# Autodesk Inventor assembly: bottomLayer
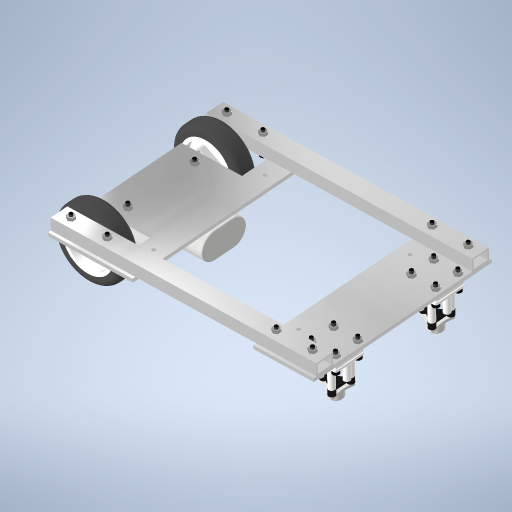
[picture p0: Inventor's stored thumbnail of the model, 512x512]
Saved by Autodesk Inventor 2024 (Build 280153000, 153)
## iProperties
Created: 2023-10-26
Part Number: bottomLayer
Document SubType Name: Assembly
Designer: jwith
Mass: 389.888 g
Surface Area: 1411.33 cm^2
Volume: 227.835 cm^3
Density: 1.71127 g/cm^3
Author: jwith
## Documents named in this file (14)
- C:\Users\jwith\OneDrive\kikaiken\inventor\general-useLandRobotV1\bottomLayer.iam
- C:\Users\jwith\OneDrive\kikaiken\inventor\general-useLandRobotV1\backPlate.ipt
- C:\Users\jwith\OneDrive\kikaiken\inventor\general-useLandRobotV1\frontPlate.ipt
- C:\Users\jwith\OneDrive\kikaiken\inventor\general-useLandRobotV1\right_ASP.ipt
- C:\Users\jwith\OneDrive\kikaiken\inventor\general-useLandRobotV1\left_ASP.ipt
- C:\Users\jwith\OneDrive\kikaiken\inventor\general-useLandRobotV1\Content Center Files\R2024\ja-JP\SpringWasher\SpringWasher_3007SL.ipt
- C:\Users\jwith\OneDrive\kikaiken\inventor\general-useLandRobotV1\Content Center Files\R2024\ja-JP\HexSocketCapScrew\HexSocketCapScrew_3005018BK.ipt
- C:\Users\jwith\OneDrive\kikaiken\inventor\general-useLandRobotV1\Content Center Files\R2024\ja-JP\HexNut_Type1\HexNut_Type1_30050SL.ipt
- C:\Users\jwith\OneDrive\kikaiken\inventor\general-useLandRobotV1\資料\車体設計例\plate_5mm.ipt
- C:\Users\jwith\OneDrive\kikaiken\inventor\general-useLandRobotV1\資料\車体設計例\TAMIYA_ballcaster_35mm.iam
- C:\Users\jwith\OneDrive\kikaiken\inventor\general-useLandRobotV1\Content Center Files\R2024\ja-JP\HexSocketCapScrew\HexSocketCapScrew_3005015BK.ipt
- C:\Users\jwith\OneDrive\kikaiken\inventor\general-useLandRobotV1\資料\車体設計例\TAMIYA_DoubleGearBox.iam
- C:\Users\jwith\OneDrive\kikaiken\inventor\general-useLandRobotV1\Content Center Files\R2024\ja-JP\HexSocketCapScrew\HexSocketCapScrew_3005010BK.ipt
- C:\Users\jwith\OneDrive\kikaiken\inventor\general-useLandRobotV1\資料\車体設計例\ナロータイヤセット.iam
## Components (56 placed, 13 different names)
1. backPlate:1 — 回転:25, メイト:68, 回転:26, 回転:27, 回転:28, 回転:29, 回転:30, メイト:69, メイト:70, メイト:71, メイト:73, メイト:74, メイト:75, メイト:80, メイト:81, メイト:82, メイト:83, メイト:85, メイト:86, メイト:87
2. frontPlate:1 — 回転:1, 回転:2, 回転:5, 回転:6, メイト:1, メイト:2, メイト:3, メイト:5, メイト:6, メイト:7, メイト:25, メイト:26, メイト:27, メイト:29, メイト:30, メイト:31, 回転:9, 回転:10, 回転:11, 回転:12, 回転:13, 回転:14, 回転:15, 回転:16, メイト:36, メイト:40, メイト:44, メイト:48, メイト:52, メイト:56, メイト:60, メイト:64
3. right_ASP:1 — 回転:5, 回転:6, メイト:28, メイト:32, 回転:26, 回転:27, メイト:72, メイト:76
4. left_ASP:1 — 回転:1, 回転:2, メイト:4, メイト:8, 回転:28, 回転:29, メイト:84, メイト:88
5. SpringWasher M3-1.1:1 — メイト:1, メイト:2, 挿入:1
6. HexSocketCapScrew M3x0.5-18:1 — 挿入:1
7. HexNut_Type1 M3x0.5:1 — メイト:3, メイト:4
8. SpringWasher M3-1.1:2 — メイト:5, メイト:6, 挿入:2
9. HexSocketCapScrew M3x0.5-18:2 — 挿入:2
10. HexNut_Type1 M3x0.5:2 — メイト:7, メイト:8
11. SpringWasher M3-1.1:7 — メイト:25, メイト:26, 挿入:7
12. HexSocketCapScrew M3x0.5-18:7 — 挿入:7
13. HexNut_Type1 M3x0.5:7 — メイト:27, メイト:28
14. SpringWasher M3-1.1:8 — メイト:29, メイト:30, 挿入:8
15. HexSocketCapScrew M3x0.5-18:8 — 挿入:8
16. HexNut_Type1 M3x0.5:8 — メイト:31, メイト:32
17. plate_5mm:1 — 回転:13, 回転:14, 回転:15, 回転:16, 回転:21, 回転:22, 回転:23, 回転:24
18. plate_5mm:2 — 回転:9, 回転:10, 回転:11, 回転:12, 回転:17, 回転:18, 回転:19, 回転:20, メイト:33, メイト:35, メイト:45, メイト:47
19. TAMIYA_ballcaster_35mm:1 [sub-assembly] — 回転:17, 回転:18, 回転:19, 回転:20, メイト:34, メイト:37, メイト:38, メイト:39, メイト:41, メイト:42, メイト:43, メイト:46
20. TAMIYA_ballcaster_35mm:2 [sub-assembly] — 回転:21, 回転:22, 回転:23, 回転:24, メイト:49, メイト:50, メイト:51, メイト:53, メイト:54, メイト:55, メイト:57, メイト:58, メイト:59, メイト:61, メイト:62, メイト:63
21. HexSocketCapScrew M3x0.5-15:1 — メイト:33, メイト:34
22. HexNut_Type1 M3x0.5:9 — メイト:35, メイト:36
23. HexSocketCapScrew M3x0.5-15:2 — メイト:37, メイト:38
24. HexNut_Type1 M3x0.5:10 — メイト:39, メイト:40
25. HexSocketCapScrew M3x0.5-15:3 — メイト:41, メイト:42
26. HexNut_Type1 M3x0.5:11 — メイト:43, メイト:44
27. HexSocketCapScrew M3x0.5-15:4 — メイト:45, メイト:46
28. HexNut_Type1 M3x0.5:12 — メイト:47, メイト:48
29. HexSocketCapScrew M3x0.5-15:5 — メイト:49, メイト:50
30. HexNut_Type1 M3x0.5:13 — メイト:51, メイト:52
31. HexSocketCapScrew M3x0.5-15:6 — メイト:53, メイト:54
32. HexNut_Type1 M3x0.5:14 — メイト:55, メイト:56
33. HexSocketCapScrew M3x0.5-15:7 — メイト:57, メイト:58
34. HexNut_Type1 M3x0.5:15 — メイト:59, メイト:60
35. HexSocketCapScrew M3x0.5-15:8 — メイト:61, メイト:62
36. HexNut_Type1 M3x0.5:16 — メイト:63, メイト:64
37. TAMIYA_DoubleGearBox:1 [sub-assembly] — 回転:25, メイト:65, メイト:66, メイト:67, リジッド:1, 回転:30, メイト:77, メイト:78, メイト:79, リジッド:2
38. HexSocketCapScrew M3x0.5-10:1 — メイト:65, メイト:66
39. HexNut_Type1 M3x0.5:17 — メイト:67, メイト:68
40. ナロータイヤセット:1 [sub-assembly] — リジッド:1
41. SpringWasher M3-1.1:9 — メイト:69, メイト:70, 挿入:9
42. HexSocketCapScrew M3x0.5-18:9 — 挿入:9
43. HexNut_Type1 M3x0.5:18 — メイト:71, メイト:72
44. SpringWasher M3-1.1:10 — メイト:73, メイト:74, 挿入:10
45. HexSocketCapScrew M3x0.5-18:10 — 挿入:10
46. HexNut_Type1 M3x0.5:19 — メイト:75, メイト:76
47. SpringWasher M3-1.1:11 — メイト:77, メイト:78, 挿入:11
48. HexSocketCapScrew M3x0.5-10:2 — 挿入:11
49. HexNut_Type1 M3x0.5:20 — メイト:79, メイト:80
50. SpringWasher M3-1.1:12 — メイト:81, メイト:82, 挿入:12
51. HexSocketCapScrew M3x0.5-18:11 — 挿入:12
52. HexNut_Type1 M3x0.5:21 — メイト:83, メイト:84
53. SpringWasher M3-1.1:13 — メイト:85, メイト:86, 挿入:13
54. HexSocketCapScrew M3x0.5-18:12 — 挿入:13
55. HexNut_Type1 M3x0.5:22 — メイト:87, メイト:88
56. ナロータイヤセット:2 [sub-assembly] — リジッド:2
## Relationships (109: Mate 72, RevoluteJoint 26, Insert 9, WeldJoint 2)
- 回転:1 [RevoluteJoint]: frontPlate:1 ↔ left_ASP:1
- 回転:2 [RevoluteJoint]: frontPlate:1 ↔ left_ASP:1
- 回転:5 [RevoluteJoint]: frontPlate:1 ↔ right_ASP:1
- 回転:6 [RevoluteJoint]: frontPlate:1 ↔ right_ASP:1
- メイト:1 [Mate]: frontPlate:1 ↔ SpringWasher M3-1.1:1
- メイト:2 [Mate]: frontPlate:1 ↔ SpringWasher M3-1.1:1
- 挿入:1 [Insert]: SpringWasher M3-1.1:1 ↔ HexSocketCapScrew M3x0.5-18:1
- メイト:3 [Mate]: frontPlate:1 ↔ HexNut_Type1 M3x0.5:1
- メイト:4 [Mate]: left_ASP:1 ↔ HexNut_Type1 M3x0.5:1
- メイト:5 [Mate]: frontPlate:1 ↔ SpringWasher M3-1.1:2
- メイト:6 [Mate]: frontPlate:1 ↔ SpringWasher M3-1.1:2
- 挿入:2 [Insert]: SpringWasher M3-1.1:2 ↔ HexSocketCapScrew M3x0.5-18:2
- メイト:7 [Mate]: frontPlate:1 ↔ HexNut_Type1 M3x0.5:2
- メイト:8 [Mate]: left_ASP:1 ↔ HexNut_Type1 M3x0.5:2
- メイト:25 [Mate]: frontPlate:1 ↔ SpringWasher M3-1.1:7
- メイト:26 [Mate]: frontPlate:1 ↔ SpringWasher M3-1.1:7
- 挿入:7 [Insert]: SpringWasher M3-1.1:7 ↔ HexSocketCapScrew M3x0.5-18:7
- メイト:27 [Mate]: frontPlate:1 ↔ HexNut_Type1 M3x0.5:7
- メイト:28 [Mate]: right_ASP:1 ↔ HexNut_Type1 M3x0.5:7
- メイト:29 [Mate]: frontPlate:1 ↔ SpringWasher M3-1.1:8
- メイト:30 [Mate]: frontPlate:1 ↔ SpringWasher M3-1.1:8
- 挿入:8 [Insert]: SpringWasher M3-1.1:8 ↔ HexSocketCapScrew M3x0.5-18:8
- メイト:31 [Mate]: frontPlate:1 ↔ HexNut_Type1 M3x0.5:8
- メイト:32 [Mate]: right_ASP:1 ↔ HexNut_Type1 M3x0.5:8
- 回転:9 [RevoluteJoint]: frontPlate:1 ↔ plate_5mm:2
- 回転:10 [RevoluteJoint]: frontPlate:1 ↔ plate_5mm:2
- 回転:11 [RevoluteJoint]: frontPlate:1 ↔ plate_5mm:2
- 回転:12 [RevoluteJoint]: frontPlate:1 ↔ plate_5mm:2
- 回転:13 [RevoluteJoint]: frontPlate:1 ↔ plate_5mm:1
- 回転:14 [RevoluteJoint]: frontPlate:1 ↔ plate_5mm:1
- 回転:15 [RevoluteJoint]: frontPlate:1 ↔ plate_5mm:1
- 回転:16 [RevoluteJoint]: frontPlate:1 ↔ plate_5mm:1
- 回転:17 [RevoluteJoint]: plate_5mm:2 ↔ TAMIYA_ballcaster_35mm:1
- 回転:18 [RevoluteJoint]: plate_5mm:2 ↔ TAMIYA_ballcaster_35mm:1
- 回転:19 [RevoluteJoint]: plate_5mm:2 ↔ TAMIYA_ballcaster_35mm:1
- 回転:20 [RevoluteJoint]: plate_5mm:2 ↔ TAMIYA_ballcaster_35mm:1
- 回転:21 [RevoluteJoint]: plate_5mm:1 ↔ TAMIYA_ballcaster_35mm:2
- 回転:22 [RevoluteJoint]: plate_5mm:1 ↔ TAMIYA_ballcaster_35mm:2
- 回転:23 [RevoluteJoint]: plate_5mm:1 ↔ TAMIYA_ballcaster_35mm:2
- 回転:24 [RevoluteJoint]: plate_5mm:1 ↔ TAMIYA_ballcaster_35mm:2
- メイト:33 [Mate]: plate_5mm:2 ↔ HexSocketCapScrew M3x0.5-15:1
- メイト:34 [Mate]: TAMIYA_ballcaster_35mm:1 ↔ HexSocketCapScrew M3x0.5-15:1
- メイト:35 [Mate]: plate_5mm:2 ↔ HexNut_Type1 M3x0.5:9
- メイト:36 [Mate]: frontPlate:1 ↔ HexNut_Type1 M3x0.5:9
- メイト:37 [Mate]: TAMIYA_ballcaster_35mm:1 ↔ HexSocketCapScrew M3x0.5-15:2
- メイト:38 [Mate]: TAMIYA_ballcaster_35mm:1 ↔ HexSocketCapScrew M3x0.5-15:2
- メイト:39 [Mate]: TAMIYA_ballcaster_35mm:1 ↔ HexNut_Type1 M3x0.5:10
- メイト:40 [Mate]: frontPlate:1 ↔ HexNut_Type1 M3x0.5:10
- メイト:41 [Mate]: TAMIYA_ballcaster_35mm:1 ↔ HexSocketCapScrew M3x0.5-15:3
- メイト:42 [Mate]: TAMIYA_ballcaster_35mm:1 ↔ HexSocketCapScrew M3x0.5-15:3
- メイト:43 [Mate]: TAMIYA_ballcaster_35mm:1 ↔ HexNut_Type1 M3x0.5:11
- メイト:44 [Mate]: frontPlate:1 ↔ HexNut_Type1 M3x0.5:11
- メイト:45 [Mate]: plate_5mm:2 ↔ HexSocketCapScrew M3x0.5-15:4
- メイト:46 [Mate]: TAMIYA_ballcaster_35mm:1 ↔ HexSocketCapScrew M3x0.5-15:4
- メイト:47 [Mate]: plate_5mm:2 ↔ HexNut_Type1 M3x0.5:12
- メイト:48 [Mate]: frontPlate:1 ↔ HexNut_Type1 M3x0.5:12
- メイト:49 [Mate]: TAMIYA_ballcaster_35mm:2 ↔ HexSocketCapScrew M3x0.5-15:5
- メイト:50 [Mate]: TAMIYA_ballcaster_35mm:2 ↔ HexSocketCapScrew M3x0.5-15:5
- メイト:51 [Mate]: TAMIYA_ballcaster_35mm:2 ↔ HexNut_Type1 M3x0.5:13
- メイト:52 [Mate]: frontPlate:1 ↔ HexNut_Type1 M3x0.5:13
- メイト:53 [Mate]: TAMIYA_ballcaster_35mm:2 ↔ HexSocketCapScrew M3x0.5-15:6
- メイト:54 [Mate]: TAMIYA_ballcaster_35mm:2 ↔ HexSocketCapScrew M3x0.5-15:6
- メイト:55 [Mate]: TAMIYA_ballcaster_35mm:2 ↔ HexNut_Type1 M3x0.5:14
- メイト:56 [Mate]: frontPlate:1 ↔ HexNut_Type1 M3x0.5:14
- メイト:57 [Mate]: TAMIYA_ballcaster_35mm:2 ↔ HexSocketCapScrew M3x0.5-15:7
- メイト:58 [Mate]: TAMIYA_ballcaster_35mm:2 ↔ HexSocketCapScrew M3x0.5-15:7
- メイト:59 [Mate]: TAMIYA_ballcaster_35mm:2 ↔ HexNut_Type1 M3x0.5:15
- メイト:60 [Mate]: frontPlate:1 ↔ HexNut_Type1 M3x0.5:15
- メイト:61 [Mate]: TAMIYA_ballcaster_35mm:2 ↔ HexSocketCapScrew M3x0.5-15:8
- メイト:62 [Mate]: TAMIYA_ballcaster_35mm:2 ↔ HexSocketCapScrew M3x0.5-15:8
- メイト:63 [Mate]: TAMIYA_ballcaster_35mm:2 ↔ HexNut_Type1 M3x0.5:16
- メイト:64 [Mate]: frontPlate:1 ↔ HexNut_Type1 M3x0.5:16
- 回転:25 [RevoluteJoint]: backPlate:1 ↔ TAMIYA_DoubleGearBox:1
- メイト:65 [Mate]: TAMIYA_DoubleGearBox:1 ↔ HexSocketCapScrew M3x0.5-10:1
- メイト:66 [Mate]: TAMIYA_DoubleGearBox:1 ↔ HexSocketCapScrew M3x0.5-10:1
- メイト:67 [Mate]: TAMIYA_DoubleGearBox:1 ↔ HexNut_Type1 M3x0.5:17
- メイト:68 [Mate]: backPlate:1 ↔ HexNut_Type1 M3x0.5:17
- リジッド:1 [WeldJoint]: TAMIYA_DoubleGearBox:1 ↔ ナロータイヤセット:1
- 回転:26 [RevoluteJoint]: backPlate:1 ↔ right_ASP:1
- 回転:27 [RevoluteJoint]: backPlate:1 ↔ right_ASP:1
- 回転:28 [RevoluteJoint]: backPlate:1 ↔ left_ASP:1
- 回転:29 [RevoluteJoint]: backPlate:1 ↔ left_ASP:1
- 回転:30 [RevoluteJoint]: backPlate:1 ↔ TAMIYA_DoubleGearBox:1
- メイト:69 [Mate]: backPlate:1 ↔ SpringWasher M3-1.1:9
- メイト:70 [Mate]: backPlate:1 ↔ SpringWasher M3-1.1:9
- 挿入:9 [Insert]: SpringWasher M3-1.1:9 ↔ HexSocketCapScrew M3x0.5-18:9
- メイト:71 [Mate]: backPlate:1 ↔ HexNut_Type1 M3x0.5:18
- メイト:72 [Mate]: right_ASP:1 ↔ HexNut_Type1 M3x0.5:18
- メイト:73 [Mate]: backPlate:1 ↔ SpringWasher M3-1.1:10
- メイト:74 [Mate]: backPlate:1 ↔ SpringWasher M3-1.1:10
- 挿入:10 [Insert]: SpringWasher M3-1.1:10 ↔ HexSocketCapScrew M3x0.5-18:10
- メイト:75 [Mate]: backPlate:1 ↔ HexNut_Type1 M3x0.5:19
- メイト:76 [Mate]: right_ASP:1 ↔ HexNut_Type1 M3x0.5:19
- メイト:77 [Mate]: TAMIYA_DoubleGearBox:1 ↔ SpringWasher M3-1.1:11
- メイト:78 [Mate]: TAMIYA_DoubleGearBox:1 ↔ SpringWasher M3-1.1:11
- 挿入:11 [Insert]: SpringWasher M3-1.1:11 ↔ HexSocketCapScrew M3x0.5-10:2
- メイト:79 [Mate]: TAMIYA_DoubleGearBox:1 ↔ HexNut_Type1 M3x0.5:20
- メイト:80 [Mate]: backPlate:1 ↔ HexNut_Type1 M3x0.5:20
- メイト:81 [Mate]: backPlate:1 ↔ SpringWasher M3-1.1:12
- メイト:82 [Mate]: backPlate:1 ↔ SpringWasher M3-1.1:12
- 挿入:12 [Insert]: SpringWasher M3-1.1:12 ↔ HexSocketCapScrew M3x0.5-18:11
- メイト:83 [Mate]: backPlate:1 ↔ HexNut_Type1 M3x0.5:21
- メイト:84 [Mate]: left_ASP:1 ↔ HexNut_Type1 M3x0.5:21
- メイト:85 [Mate]: backPlate:1 ↔ SpringWasher M3-1.1:13
- メイト:86 [Mate]: backPlate:1 ↔ SpringWasher M3-1.1:13
- 挿入:13 [Insert]: SpringWasher M3-1.1:13 ↔ HexSocketCapScrew M3x0.5-18:12
- メイト:87 [Mate]: backPlate:1 ↔ HexNut_Type1 M3x0.5:22
- メイト:88 [Mate]: left_ASP:1 ↔ HexNut_Type1 M3x0.5:22
- リジッド:2 [WeldJoint]: TAMIYA_DoubleGearBox:1 ↔ ナロータイヤセット:2
